# Autodesk Inventor assembly: origami
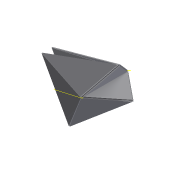
[picture p0: Inventor's stored thumbnail of the model, 180x180]
Saved by Autodesk Inventor 2019.4 (Build 234330000, 330)
## iProperties
Created: 2018-08-06
Part Number: origami
Material: 一般
Document SubType Name: Assembly
Designer: AzLIer
Author: AzLIer
## Documents named in this file (4)
- E:\ロボ研\キャチロボ\キャチロボ2018\アーム\アーム01\hand02\origami.iam
- E:\ロボ研\キャチロボ\キャチロボ2018\アーム\アーム01\hand02\origami01.ipt
- E:\ロボ研\キャチロボ\キャチロボ2018\アーム\アーム01\hand02\origami02.ipt
- E:\ロボ研\キャチロボ\キャチロボ2018\アーム\アーム01\hand02\origami03.ipt
## Components (8 placed, 3 different names)
1. origami01:1 — 回転:1, 回転:5, 回転:7, フラッシュ:1, メイト:1
2. origami02:1 — 回転:1, 回転:2, 角度:2
3. origami03:1 — 回転:2, 回転:3, メイト:1, メイト:3
4. origami02:2 — 回転:3, 回転:4, 角度:1
5. origami01:2 — 回転:4, 回転:5, 回転:6, フラッシュ:1, メイト:2
6. origami02:3 — 回転:6, 回転:8, 角度:1
7. origami02:4 — 回転:7, 回転:9, 角度:2
8. origami03:2 — 回転:8, 回転:9, メイト:2, メイト:3
## Relationships (15: RevoluteJoint 9, Mate 3, Angle 2, Flush 1)
- 回転:1 [RevoluteJoint]: origami01:1 ↔ origami02:1
- 回転:2 [RevoluteJoint]: origami02:1 ↔ origami03:1
- 回転:3 [RevoluteJoint]: origami03:1 ↔ origami02:2
- 回転:4 [RevoluteJoint]: origami02:2 ↔ origami01:2
- 回転:5 [RevoluteJoint]: origami01:1 ↔ origami01:2
- 回転:6 [RevoluteJoint]: origami01:2 ↔ origami02:3
- 回転:7 [RevoluteJoint]: origami01:1 ↔ origami02:4
- 回転:8 [RevoluteJoint]: origami02:3 ↔ origami03:2
- 回転:9 [RevoluteJoint]: origami02:4 ↔ origami03:2
- フラッシュ:1 [Flush]: origami01:1 ↔ origami01:2
- 角度:1 [Angle] (0 deg): origami02:2 ↔ origami02:3
- 角度:2 [Angle] (0 deg): origami02:1 ↔ origami02:4
- メイト:1 [Mate]: origami01:1 ↔ origami03:1
- メイト:2 [Mate]: origami01:2 ↔ origami03:2
- メイト:3 [Mate] (80 mm): origami03:1 ↔ origami03:2
